(part 1 of 2)
# Autodesk Inventor assembly: Remote_Station
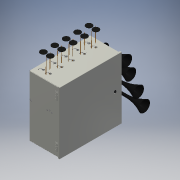
[picture p0: Inventor's stored thumbnail of the model, 180x180]
Saved by Autodesk Inventor 2016 (Build 200138000, 138)
## iProperties
Created: 2016-05-06
Part Number: Remote_Station
Document SubType Name: Assembly
Designer: agmle
Mass: 29128.1 g
Surface Area: 35809.2 cm^2
Volume: 7544.68 cm^3
Density: 3.86075 g/cm^3
Author: agmle
## Documents named in this file (30)
- C:\Users\agmle\BitTorrent Sync\private\projects\Creekfleet_Timer\hardware\CAD\Remote\Remote_Station.iam
- C:\Users\agmle\BitTorrent Sync\private\projects\Creekfleet_Timer\hardware\CAD\Remote\ASM_Winch.iam
- C:\Users\agmle\BitTorrent Sync\private\projects\Creekfleet_Timer\hardware\CAD\Remote\SCESCE-20N2010LP.ipt
- C:\Users\agmle\BitTorrent Sync\private\projects\Creekfleet_Timer\hardware\CAD\Remote\RSF 46-1M_NPT.ipt
- C:\Users\agmle\BitTorrent Sync\private\projects\Creekfleet_Timer\hardware\CAD\Remote\Winch_Plate_Front.ipt
- C:\Users\agmle\Documents\Inventor\Content Center Files\R2016\en-US\ANSI B18.3(05)\ANSI B18.3 - 10-32 UNF - 0.75(31).ipt
- C:\Users\agmle\Documents\Inventor\Content Center Files\R2016\en-US\ANSI B18.22.1\ANSI B18.22.1 - No. 12 - narrow - Type B.ipt
- C:\Users\agmle\Documents\Inventor\Content Center Files\R2016\en-US\ASME B18.21.1(08)\ASME B18.21.1 - No. 12. Carbon Steel(2) A.ipt
- C:\Users\agmle\BitTorrent Sync\private\projects\Creekfleet_Timer\hardware\CAD\Remote\Winch_Plate_Rear.ipt
- C:\Users\agmle\BitTorrent Sync\private\projects\Creekfleet_Timer\hardware\CAD\Remote\Deck_Bushing.iam
- C:\Users\agmle\BitTorrent Sync\private\projects\Creekfleet_Timer\hardware\CAD\Remote\Fender.ipt
- C:\Users\agmle\BitTorrent Sync\private\projects\Creekfleet_Timer\hardware\CAD\Remote\Cherry_KWBH0001\KWBH0001.iam
- C:\Users\agmle\BitTorrent Sync\private\projects\Creekfleet_Timer\hardware\CAD\Remote\Microswitch_Bracket.ipt
- C:\Users\agmle\Documents\Inventor\Content Center Files\R2016\en-US\ASME B18.21.1(08)\ASME B18.21.1 - No. 4. Carbon Steel(2) A.ipt
- C:\Users\agmle\Documents\Inventor\Content Center Files\R2016\en-US\ANSI B18.22.1\ANSI B18.22.1 - No. 4 - narrow - Type B.ipt
- C:\Users\agmle\Documents\Inventor\Content Center Files\R2016\en-US\ANSI B18.3(03)\ANSI B18.3 - 4-40 UNC - UNC - 0.75(1).ipt
- C:\Users\agmle\BitTorrent Sync\private\projects\Creekfleet_Timer\hardware\CAD\Main\9414K360.ipt
- C:\Users\agmle\BitTorrent Sync\private\projects\Creekfleet_Timer\hardware\CAD\Main\9414K930.ipt
- C:\Users\agmle\BitTorrent Sync\private\projects\Creekfleet_Timer\hardware\CAD\Remote\Cap_Mount.ipt
- C:\Users\agmle\BitTorrent Sync\private\projects\Creekfleet_Timer\hardware\CAD\Remote\3.5F_Cap.ipt
- C:\Users\agmle\Documents\Inventor\Content Center Files\R2016\en-US\ANSI B18.3(04)\ANSI B18.3 - 4-40 UNC - 0.25(30).ipt
- C:\Users\agmle\Documents\Inventor\Content Center Files\R2016\en-US\ANSI B18.6.3(36)\ANSI B18.6.3 - 10 - 32(2).ipt
- C:\Users\agmle\BitTorrent Sync\private\projects\Creekfleet_Timer\hardware\CAD\Remote\Horn.iam
- C:\Users\agmle\Documents\Inventor\Content Center Files\R2016\en-US\ANSI B 18.2.4.1 M(1)\ANSI B 18.2.4.1 M - M8 x 1.25Style 1.ipt
- C:\Users\agmle\Documents\Inventor\Content Center Files\R2016\en-US\ANSI B18.22 M\ANSI B18.22M - 8 N.ipt
- C:\Users\agmle\Documents\Inventor\Content Center Files\R2016\en-US\ANSI B18.21.1\ANSI B18.21.1 - 0.375.ipt
- C:\Users\agmle\Documents\Inventor\Content Center Files\R2016\en-US\ANSI B18.2.3.5M\ANSI B18.2.3.5M - M8 x 1.25 x 30.ipt
- C:\Users\agmle\BitTorrent Sync\private\projects\Creekfleet_Timer\hardware\CAD\Remote\Barrel_Jack.ipt
- C:\Users\agmle\BitTorrent Sync\private\projects\Creekfleet_Timer\hardware\CAD\Remote\Norgren-R07-100-RGEA+18-025-003+18-013-212.iam
- C:\Users\agmle\Documents\Inventor\Content Center Files\R2016\en-US\ANSI B18.3(05)\ANSI B18.3 - 10-32 UNF - 0.5(31).ipt
## Components (337 placed, 29 different names)
1. ASM_Winch:1 [sub-assembly] — Insert:6, Insert:7, Insert:93
2. ASM_Winch:2 [sub-assembly] — Insert:5, Insert:8
3. ASM_Winch:3 [sub-assembly] — Insert:4, Insert:9
4. ASM_Winch:4 [sub-assembly] — Insert:3, Insert:10
5. ASM_Winch:5 [sub-assembly] — Insert:2, Insert:11, Insert:92
6. SCESCE-20N2010LP:1 — Insert:1, Insert:12, Insert:13, Insert:26, Insert:27, Insert:28, Insert:29, Insert:30, Insert:31, Insert:98, Insert:99, Insert:104, Insert:105, Insert:106, Insert:107, Insert:108, Insert:109, Insert:110, Insert:111, Insert:112, Insert:113, Insert:114, Insert:115, Mate:1, Mate:2, Mate:3, Mate:4, Mate:5, Mate:6, Mate:7, Mate:8, Mate:9, Mate:10, Mate:11, Mate:12, Flush:1, Mate:14, Angle:1, Mate:16, Mate:17, Insert:147, Insert:148, Mate:18, Mate:19, Mate:20, Mate:21, Mate:22, Mate:23, Mate:24, Mate:25, Mate:26, Mate:27, Mate:28, Mate:29, Mate:30, Mate:31, Mate:32, Mate:33, Mate:34, Mate:35, Insert:248, Insert:249, Insert:250, Insert:251, Insert:252, Insert:253, Insert:254, Insert:255, Insert:256, Insert:257, Insert:258, Insert:259, Insert:260, Insert:261, Insert:262, Insert:263, Insert:264, Insert:265, Insert:267, Insert:268, Insert:269, Insert:286, Insert:287, Insert:288, Insert:289, Insert:294, Mate:47, Insert:304, Insert:305, Insert:306, Insert:307, Mate:48, Insert:308, Tangent:1, Insert:319, Insert:320, Insert:322
7. RSF 46-1M_NPT:1 — Insert:1
8. Winch_Plate_Front:1 — Insert:2, Insert:3, Insert:4, Insert:5, Insert:6, Insert:7, Insert:8, Insert:9, Insert:10, Insert:11, Insert:12, Insert:13, Insert:72, Insert:73, Insert:74, Insert:75, Insert:76, Insert:77, Insert:78, Insert:79, Insert:80, Insert:81, Insert:82, Insert:83, Insert:84, Insert:85, Insert:86, Insert:87, Insert:88, Insert:89, Insert:90, Insert:91
9. Hexagon Socket Head Cap Screw - Inch 10-32 UNF - 0.75:5 — Insert:14
10. Plain Washer (Inch) No. 12 - narrow - Type B:1 — Insert:15, Insert:27
11. Internal Tooth Lock Washer - Type A (Inch) No. 12. Carbon Steel:1 — Insert:14, Insert:15
12. Hexagon Socket Head Cap Screw - Inch 10-32 UNF - 0.75:6
13. Plain Washer (Inch) No. 12 - narrow - Type B:2 — Insert:29
14. Internal Tooth Lock Washer - Type A (Inch) No. 12. Carbon Steel:2
15. Hexagon Socket Head Cap Screw - Inch 10-32 UNF - 0.75:7
16. Plain Washer (Inch) No. 12 - narrow - Type B:3 — Insert:30
17. Internal Tooth Lock Washer - Type A (Inch) No. 12. Carbon Steel:3
18. Hexagon Socket Head Cap Screw - Inch 10-32 UNF - 0.75:8
19. Plain Washer (Inch) No. 12 - narrow - Type B:4 — Insert:26
20. Internal Tooth Lock Washer - Type A (Inch) No. 12. Carbon Steel:4
21. Hexagon Socket Head Cap Screw - Inch 10-32 UNF - 0.75:9
22. Plain Washer (Inch) No. 12 - narrow - Type B:5 — Insert:28
23. Internal Tooth Lock Washer - Type A (Inch) No. 12. Carbon Steel:5
24. Hexagon Socket Head Cap Screw - Inch 10-32 UNF - 0.75:10
25. Plain Washer (Inch) No. 12 - narrow - Type B:6 — Insert:31
26. Internal Tooth Lock Washer - Type A (Inch) No. 12. Carbon Steel:6
27. Hexagon Socket Head Cap Screw - Inch 10-32 UNF - 0.75:11
28. Plain Washer (Inch) No. 12 - narrow - Type B:7 — Insert:72
29. Internal Tooth Lock Washer - Type A (Inch) No. 12. Carbon Steel:7
30. Hexagon Socket Head Cap Screw - Inch 10-32 UNF - 0.75:12
31. Plain Washer (Inch) No. 12 - narrow - Type B:8 — Insert:73
32. Internal Tooth Lock Washer - Type A (Inch) No. 12. Carbon Steel:8
33. Hexagon Socket Head Cap Screw - Inch 10-32 UNF - 0.75:13
34. Plain Washer (Inch) No. 12 - narrow - Type B:9 — Insert:75
35. Internal Tooth Lock Washer - Type A (Inch) No. 12. Carbon Steel:9
36. Hexagon Socket Head Cap Screw - Inch 10-32 UNF - 0.75:14
37. Plain Washer (Inch) No. 12 - narrow - Type B:10 — Insert:74
38. Internal Tooth Lock Washer - Type A (Inch) No. 12. Carbon Steel:10
39. Hexagon Socket Head Cap Screw - Inch 10-32 UNF - 0.75:15
40. Plain Washer (Inch) No. 12 - narrow - Type B:11 — Insert:76
41. Internal Tooth Lock Washer - Type A (Inch) No. 12. Carbon Steel:11
42. Hexagon Socket Head Cap Screw - Inch 10-32 UNF - 0.75:16
43. Plain Washer (Inch) No. 12 - narrow - Type B:12 — Insert:78
44. Internal Tooth Lock Washer - Type A (Inch) No. 12. Carbon Steel:12
45. Hexagon Socket Head Cap Screw - Inch 10-32 UNF - 0.75:17
46. Plain Washer (Inch) No. 12 - narrow - Type B:13 — Insert:79
47. Internal Tooth Lock Washer - Type A (Inch) No. 12. Carbon Steel:13
48. Hexagon Socket Head Cap Screw - Inch 10-32 UNF - 0.75:18
49. Plain Washer (Inch) No. 12 - narrow - Type B:14 — Insert:77
50. Internal Tooth Lock Washer - Type A (Inch) No. 12. Carbon Steel:14
51. Hexagon Socket Head Cap Screw - Inch 10-32 UNF - 0.75:19
52. Plain Washer (Inch) No. 12 - narrow - Type B:15 — Insert:80
53. Internal Tooth Lock Washer - Type A (Inch) No. 12. Carbon Steel:15
54. Hexagon Socket Head Cap Screw - Inch 10-32 UNF - 0.75:20
55. Plain Washer (Inch) No. 12 - narrow - Type B:16 — Insert:81
56. Internal Tooth Lock Washer - Type A (Inch) No. 12. Carbon Steel:16
57. Hexagon Socket Head Cap Screw - Inch 10-32 UNF - 0.75:21
58. Plain Washer (Inch) No. 12 - narrow - Type B:17 — Insert:82
59. Internal Tooth Lock Washer - Type A (Inch) No. 12. Carbon Steel:17
60. Hexagon Socket Head Cap Screw - Inch 10-32 UNF - 0.75:22
61. Plain Washer (Inch) No. 12 - narrow - Type B:18 — Insert:83
62. Internal Tooth Lock Washer - Type A (Inch) No. 12. Carbon Steel:18
63. Hexagon Socket Head Cap Screw - Inch 10-32 UNF - 0.75:23
64. Plain Washer (Inch) No. 12 - narrow - Type B:19 — Insert:84
65. Internal Tooth Lock Washer - Type A (Inch) No. 12. Carbon Steel:19
66. Hexagon Socket Head Cap Screw - Inch 10-32 UNF - 0.75:24
67. Plain Washer (Inch) No. 12 - narrow - Type B:20 — Insert:85
68. Internal Tooth Lock Washer - Type A (Inch) No. 12. Carbon Steel:20
69. Hexagon Socket Head Cap Screw - Inch 10-32 UNF - 0.75:25
70. Plain Washer (Inch) No. 12 - narrow - Type B:21 — Insert:86
71. Internal Tooth Lock Washer - Type A (Inch) No. 12. Carbon Steel:21
72. Hexagon Socket Head Cap Screw - Inch 10-32 UNF - 0.75:26
73. Plain Washer (Inch) No. 12 - narrow - Type B:22 — Insert:87
74. Internal Tooth Lock Washer - Type A (Inch) No. 12. Carbon Steel:22
75. Hexagon Socket Head Cap Screw - Inch 10-32 UNF - 0.75:27
76. Plain Washer (Inch) No. 12 - narrow - Type B:23 — Insert:88
77. Internal Tooth Lock Washer - Type A (Inch) No. 12. Carbon Steel:23
78. Hexagon Socket Head Cap Screw - Inch 10-32 UNF - 0.75:28
79. Plain Washer (Inch) No. 12 - narrow - Type B:24 — Insert:89
80. Internal Tooth Lock Washer - Type A (Inch) No. 12. Carbon Steel:24
81. Hexagon Socket Head Cap Screw - Inch 10-32 UNF - 0.75:29
82. Plain Washer (Inch) No. 12 - narrow - Type B:25 — Insert:90
83. Internal Tooth Lock Washer - Type A (Inch) No. 12. Carbon Steel:25
84. Hexagon Socket Head Cap Screw - Inch 10-32 UNF - 0.75:30
85. Plain Washer (Inch) No. 12 - narrow - Type B:26 — Insert:91
86. Internal Tooth Lock Washer - Type A (Inch) No. 12. Carbon Steel:26
87. Winch_Plate_Rear:1 — Insert:92, Insert:93
88. Hexagon Socket Head Cap Screw - Inch 10-32 UNF - 0.75:31
89. Plain Washer (Inch) No. 12 - narrow - Type B:27 — Insert:98
90. Internal Tooth Lock Washer - Type A (Inch) No. 12. Carbon Steel:27
91. Hexagon Socket Head Cap Screw - Inch 10-32 UNF - 0.75:32
92. Plain Washer (Inch) No. 12 - narrow - Type B:28 — Insert:99
93. Internal Tooth Lock Washer - Type A (Inch) No. 12. Carbon Steel:28
94. Hexagon Socket Head Cap Screw - Inch 10-32 UNF - 0.75:33
95. Plain Washer (Inch) No. 12 - narrow - Type B:29 — Insert:104
96. Internal Tooth Lock Washer - Type A (Inch) No. 12. Carbon Steel:29
97. Hexagon Socket Head Cap Screw - Inch 10-32 UNF - 0.75:34
98. Plain Washer (Inch) No. 12 - narrow - Type B:30 — Insert:105
99. Internal Tooth Lock Washer - Type A (Inch) No. 12. Carbon Steel:30
100. Deck_Bushing:1 [sub-assembly] — Insert:109, Mate:4, Insert:128, Insert:130, Mate:38
101. Deck_Bushing:2 [sub-assembly] — Insert:110, Mate:6, Insert:125, Insert:126, Mate:40
102. Deck_Bushing:3 [sub-assembly] — Insert:107, Mate:2, Insert:132, Insert:134, Mate:36
103. Deck_Bushing:4 [sub-assembly] — Insert:114, Mate:9, Insert:116, Insert:119, Mate:43
104. Deck_Bushing:5 [sub-assembly] — Insert:115, Mate:10, Insert:117, Insert:118, Mate:44
105. Deck_Bushing:6 [sub-assembly] — Insert:111, Mate:5, Insert:124, Insert:127, Mate:39
106. Deck_Bushing:7 [sub-assembly] — Insert:113, Mate:7, Insert:121, Insert:123, Mate:41
107. Deck_Bushing:8 [sub-assembly] — Insert:112, Mate:8, Insert:120, Insert:122, Mate:42
108. Deck_Bushing:9 [sub-assembly] — Insert:106, Mate:1, Insert:133, Insert:135, Mate:13
109. Deck_Bushing:10 [sub-assembly] — Insert:108, Mate:3, Insert:129, Insert:131, Mate:37
110. Hexagon Socket Flat Countersunk Head Cap Screw - Inch 4-40 UNC x 0.25:1 — Insert:116
111. Hexagon Socket Flat Countersunk Head Cap Screw - Inch 4-40 UNC x 0.25:2 — Insert:117
112. Hexagon Socket Flat Countersunk Head Cap Screw - Inch 4-40 UNC x 0.25:3 — Insert:118
113. Hexagon Socket Flat Countersunk Head Cap Screw - Inch 4-40 UNC x 0.25:4 — Insert:120
114. Hexagon Socket Flat Countersunk Head Cap Screw - Inch 4-40 UNC x 0.25:5 — Insert:119
115. Hexagon Socket Flat Countersunk Head Cap Screw - Inch 4-40 UNC x 0.25:6 — Insert:121
116. Hexagon Socket Flat Countersunk Head Cap Screw - Inch 4-40 UNC x 0.25:7 — Insert:123
117. Hexagon Socket Flat Countersunk Head Cap Screw - Inch 4-40 UNC x 0.25:8 — Insert:122
118. Hexagon Socket Flat Countersunk Head Cap Screw - Inch 4-40 UNC x 0.25:9 — Insert:125
119. Hexagon Socket Flat Countersunk Head Cap Screw - Inch 4-40 UNC x 0.25:10 — Insert:124
120. Hexagon Socket Flat Countersunk Head Cap Screw - Inch 4-40 UNC x 0.25:11 — Insert:127
121. Hexagon Socket Flat Countersunk Head Cap Screw - Inch 4-40 UNC x 0.25:12 — Insert:126
122. Hexagon Socket Flat Countersunk Head Cap Screw - Inch 4-40 UNC x 0.25:13 — Insert:129
123. Hexagon Socket Flat Countersunk Head Cap Screw - Inch 4-40 UNC x 0.25:14 — Insert:128
124. Hexagon Socket Flat Countersunk Head Cap Screw - Inch 4-40 UNC x 0.25:15 — Insert:131
125. Hexagon Socket Flat Countersunk Head Cap Screw - Inch 4-40 UNC x 0.25:16 — Insert:130
126. Hexagon Socket Flat Countersunk Head Cap Screw - Inch 4-40 UNC x 0.25:17 — Insert:133
127. Hexagon Socket Flat Countersunk Head Cap Screw - Inch 4-40 UNC x 0.25:18 — Insert:132
128. Hexagon Socket Flat Countersunk Head Cap Screw - Inch 4-40 UNC x 0.25:19 — Insert:135
129. Hexagon Socket Flat Countersunk Head Cap Screw - Inch 4-40 UNC x 0.25:20 — Insert:134
130. Fender:1 — Mate:13, Mate:16, Flush:16
131. KWBH0001:1 [sub-assembly] — Insert:136, Flush:2, Insert:141, Insert:142
132. Microswitch_Bracket:1 — Insert:136, Flush:2, Mate:14, Angle:1, Mate:17, Flush:12
133. Plain Washer (Inch) No. 4 - narrow - Type B:1 — Insert:138, Insert:141
134. Internal Tooth Lock Washer - Type A (Inch) No. 4. Carbon Steel:1 — Insert:138
135. Hexagon Socket Button Head Cap Screw - Inch 4 - 40 - 3/4:1
136. Plain Washer (Inch) No. 4 - narrow - Type B:2 — Insert:142
137. Internal Tooth Lock Washer - Type A (Inch) No. 4. Carbon Steel:2
138. Hexagon Socket Button Head Cap Screw - Inch 4 - 40 - 3/4:2
139. Plain Washer (Inch) No. 4 - narrow - Type B:3 — Insert:147
140. Internal Tooth Lock Washer - Type A (Inch) No. 4. Carbon Steel:3
141. Hexagon Socket Button Head Cap Screw - Inch 4 - 40 - 3/4:3
142. Plain Washer (Inch) No. 4 - narrow - Type B:4 — Insert:148
143. Internal Tooth Lock Washer - Type A (Inch) No. 4. Carbon Steel:4
144. Hexagon Socket Button Head Cap Screw - Inch 4 - 40 - 3/4:4
145. KWBH0001:2 [sub-assembly]
146. Microswitch_Bracket:2 — Mate:18, Mate:29, Flush:13
147. Plain Washer (Inch) No. 4 - narrow - Type B:5
148. Internal Tooth Lock Washer - Type A (Inch) No. 4. Carbon Steel:5
149. Plain Washer (Inch) No. 4 - narrow - Type B:6
150. Internal Tooth Lock Washer - Type A (Inch) No. 4. Carbon Steel:6
151. Hexagon Socket Button Head Cap Screw - Inch 4 - 40 - 3/4:5
152. Hexagon Socket Button Head Cap Screw - Inch 4 - 40 - 3/4:6
153. Plain Washer (Inch) No. 4 - narrow - Type B:7 — Insert:257
154. Internal Tooth Lock Washer - Type A (Inch) No. 4. Carbon Steel:7
155. Hexagon Socket Button Head Cap Screw - Inch 4 - 40 - 3/4:7
156. Plain Washer (Inch) No. 4 - narrow - Type B:8 — Insert:252
157. Internal Tooth Lock Washer - Type A (Inch) No. 4. Carbon Steel:8
158. Hexagon Socket Button Head Cap Screw - Inch 4 - 40 - 3/4:8
159. KWBH0001:3 [sub-assembly]
160. Microswitch_Bracket:3 — Mate:22, Mate:30, Flush:14
161. Plain Washer (Inch) No. 4 - narrow - Type B:9
162. Internal Tooth Lock Washer - Type A (Inch) No. 4. Carbon Steel:9
163. Plain Washer (Inch) No. 4 - narrow - Type B:10
164. Internal Tooth Lock Washer - Type A (Inch) No. 4. Carbon Steel:10
165. Hexagon Socket Button Head Cap Screw - Inch 4 - 40 - 3/4:9
166. Hexagon Socket Button Head Cap Screw - Inch 4 - 40 - 3/4:10
167. Plain Washer (Inch) No. 4 - narrow - Type B:11 — Insert:258
168. Internal Tooth Lock Washer - Type A (Inch) No. 4. Carbon Steel:11
169. Hexagon Socket Button Head Cap Screw - Inch 4 - 40 - 3/4:11
170. Plain Washer (Inch) No. 4 - narrow - Type B:12 — Insert:256
171. Internal Tooth Lock Washer - Type A (Inch) No. 4. Carbon Steel:12
172. Hexagon Socket Button Head Cap Screw - Inch 4 - 40 - 3/4:12
173. KWBH0001:4 [sub-assembly]
174. Microswitch_Bracket:4 — Mate:24, Mate:33, Flush:15
175. Plain Washer (Inch) No. 4 - narrow - Type B:13
176. Internal Tooth Lock Washer - Type A (Inch) No. 4. Carbon Steel:13
177. Plain Washer (Inch) No. 4 - narrow - Type B:14
178. Internal Tooth Lock Washer - Type A (Inch) No. 4. Carbon Steel:14
179. Hexagon Socket Button Head Cap Screw - Inch 4 - 40 - 3/4:13
180. Hexagon Socket Button Head Cap Screw - Inch 4 - 40 - 3/4:14
181. Plain Washer (Inch) No. 4 - narrow - Type B:15 — Insert:261
182. Internal Tooth Lock Washer - Type A (Inch) No. 4. Carbon Steel:15
183. Hexagon Socket Button Head Cap Screw - Inch 4 - 40 - 3/4:15
184. Plain Washer (Inch) No. 4 - narrow - Type B:16 — Insert:260
185. Internal Tooth Lock Washer - Type A (Inch) No. 4. Carbon Steel:16
186. Hexagon Socket Button Head Cap Screw - Inch 4 - 40 - 3/4:16
187. KWBH0001:5 [sub-assembly]
188. Microswitch_Bracket:5 — Mate:26, Mate:34
189. Plain Washer (Inch) No. 4 - narrow - Type B:17
190. Internal Tooth Lock Washer - Type A (Inch) No. 4. Carbon Steel:17
191. Plain Washer (Inch) No. 4 - narrow - Type B:18
192. Internal Tooth Lock Washer - Type A (Inch) No. 4. Carbon Steel:18
193. Hexagon Socket Button Head Cap Screw - Inch 4 - 40 - 3/4:17
194. Hexagon Socket Button Head Cap Screw - Inch 4 - 40 - 3/4:18
195. Plain Washer (Inch) No. 4 - narrow - Type B:19 — Insert:264
196. Internal Tooth Lock Washer - Type A (Inch) No. 4. Carbon Steel:19
197. Hexagon Socket Button Head Cap Screw - Inch 4 - 40 - 3/4:19
198. Plain Washer (Inch) No. 4 - narrow - Type B:20 — Insert:265
199. Internal Tooth Lock Washer - Type A (Inch) No. 4. Carbon Steel:20
200. Hexagon Socket Button Head Cap Screw - Inch 4 - 40 - 3/4:20
201. KWBH0001:6 [sub-assembly]
202. Microswitch_Bracket:6 — Mate:19, Mate:27, Flush:12
203. Plain Washer (Inch) No. 4 - narrow - Type B:21
204. Internal Tooth Lock Washer - Type A (Inch) No. 4. Carbon Steel:21
205. Plain Washer (Inch) No. 4 - narrow - Type B:22
206. Internal Tooth Lock Washer - Type A (Inch) No. 4. Carbon Steel:22
207. Hexagon Socket Button Head Cap Screw - Inch 4 - 40 - 3/4:21
208. Hexagon Socket Button Head Cap Screw - Inch 4 - 40 - 3/4:22
209. Plain Washer (Inch) No. 4 - narrow - Type B:23 — Insert:249
210. Internal Tooth Lock Washer - Type A (Inch) No. 4. Carbon Steel:23
211. Hexagon Socket Button Head Cap Screw - Inch 4 - 40 - 3/4:23
212. Plain Washer (Inch) No. 4 - narrow - Type B:24 — Insert:248
213. Internal Tooth Lock Washer - Type A (Inch) No. 4. Carbon Steel:24
214. Hexagon Socket Button Head Cap Screw - Inch 4 - 40 - 3/4:24
215. KWBH0001:7 [sub-assembly]
216. Microswitch_Bracket:7 — Mate:20, Mate:28, Flush:13
217. Plain Washer (Inch) No. 4 - narrow - Type B:25
218. Internal Tooth Lock Washer - Type A (Inch) No. 4. Carbon Steel:25
219. Plain Washer (Inch) No. 4 - narrow - Type B:26
220. Internal Tooth Lock Washer - Type A (Inch) No. 4. Carbon Steel:26
221. Hexagon Socket Button Head Cap Screw - Inch 4 - 40 - 3/4:25
222. Hexagon Socket Button Head Cap Screw - Inch 4 - 40 - 3/4:26
223. Plain Washer (Inch) No. 4 - narrow - Type B:27 — Insert:251
224. Internal Tooth Lock Washer - Type A (Inch) No. 4. Carbon Steel:27
225. Hexagon Socket Button Head Cap Screw - Inch 4 - 40 - 3/4:27
226. Plain Washer (Inch) No. 4 - narrow - Type B:28 — Insert:250
227. Internal Tooth Lock Washer - Type A (Inch) No. 4. Carbon Steel:28
228. Hexagon Socket Button Head Cap Screw - Inch 4 - 40 - 3/4:28
229. KWBH0001:8 [sub-assembly]
230. Microswitch_Bracket:8 — Mate:21, Mate:31, Flush:14
231. Plain Washer (Inch) No. 4 - narrow - Type B:29
232. Internal Tooth Lock Washer - Type A (Inch) No. 4. Carbon Steel:29
233. Plain Washer (Inch) No. 4 - narrow - Type B:30
234. Internal Tooth Lock Washer - Type A (Inch) No. 4. Carbon Steel:30
235. Hexagon Socket Button Head Cap Screw - Inch 4 - 40 - 3/4:29
236. Hexagon Socket Button Head Cap Screw - Inch 4 - 40 - 3/4:30
237. Plain Washer (Inch) No. 4 - narrow - Type B:31 — Insert:254
238. Internal Tooth Lock Washer - Type A (Inch) No. 4. Carbon Steel:31
239. Hexagon Socket Button Head Cap Screw - Inch 4 - 40 - 3/4:31
240. Plain Washer (Inch) No. 4 - narrow - Type B:32 — Insert:253
241. Internal Tooth Lock Washer - Type A (Inch) No. 4. Carbon Steel:32
242. Hexagon Socket Button Head Cap Screw - Inch 4 - 40 - 3/4:32
243. KWBH0001:9 [sub-assembly]
244. Microswitch_Bracket:9 — Mate:23, Mate:32, Flush:15
245. Plain Washer (Inch) No. 4 - narrow - Type B:33
246. Internal Tooth Lock Washer - Type A (Inch) No. 4. Carbon Steel:33
247. Plain Washer (Inch) No. 4 - narrow - Type B:34
248. Internal Tooth Lock Washer - Type A (Inch) No. 4. Carbon Steel:34
249. Hexagon Socket Button Head Cap Screw - Inch 4 - 40 - 3/4:33
250. Hexagon Socket Button Head Cap Screw - Inch 4 - 40 - 3/4:34
251. Plain Washer (Inch) No. 4 - narrow - Type B:35 — Insert:259
252. Internal Tooth Lock Washer - Type A (Inch) No. 4. Carbon Steel:35
253. Hexagon Socket Button Head Cap Screw - Inch 4 - 40 - 3/4:35
254. Plain Washer (Inch) No. 4 - narrow - Type B:36 — Insert:255
255. Internal Tooth Lock Washer - Type A (Inch) No. 4. Carbon Steel:36
256. Hexagon Socket Button Head Cap Screw - Inch 4 - 40 - 3/4:36
257. KWBH0001:10 [sub-assembly]
258. Microswitch_Bracket:10 — Mate:25, Mate:35
259. Plain Washer (Inch) No. 4 - narrow - Type B:37
260. Internal Tooth Lock Washer - Type A (Inch) No. 4. Carbon Steel:37
261. Plain Washer (Inch) No. 4 - narrow - Type B:38
262. Internal Tooth Lock Washer - Type A (Inch) No. 4. Carbon Steel:38
263. Hexagon Socket Button Head Cap Screw - Inch 4 - 40 - 3/4:37
264. Hexagon Socket Button Head Cap Screw - Inch 4 - 40 - 3/4:38
265. Plain Washer (Inch) No. 4 - narrow - Type B:39 — Insert:263
266. Internal Tooth Lock Washer - Type A (Inch) No. 4. Carbon Steel:39
267. Hexagon Socket Button Head Cap Screw - Inch 4 - 40 - 3/4:39
268. Plain Washer (Inch) No. 4 - narrow - Type B:40 — Insert:262
269. Internal Tooth Lock Washer - Type A (Inch) No. 4. Carbon Steel:40
270. Hexagon Socket Button Head Cap Screw - Inch 4 - 40 - 3/4:40
271. Fender:2 — Mate:39, Flush:17, Flush:18
272. Fender:3 — Mate:40, Flush:22, Flush:23
273. Fender:4 — Mate:41, Flush:18, Flush:19
274. Fender:5 — Mate:43, Flush:19, Flush:20
275. Fender:6 — Mate:36, Flush:24
276. Fender:7 — Mate:37, Flush:16, Flush:17
277. Fender:8 — Mate:38, Flush:23, Flush:24
278. Fender:9 — Mate:42, Flush:21, Flush:22
279. Fender:10 — Mate:44, Flush:20, Flush:21
280. 9414K360:1 — Insert:266
281. 9414K930:1 — Insert:266, Insert:267
282. Cap_Mount:1 — Mate:46, Insert:268, Insert:280, Insert:281
283. Cap_Mount:2 — Mate:45, Insert:269, Insert:278, Insert:279, Flush:25
284. 3.5F_Cap:1 — Mate:45, Mate:46, Flush:25
285. Hexagon Socket Head Cap Screw - Inch 10-32 UNF - 0.5:6
286. Plain Washer (Inch) No. 12 - narrow - Type B:31 — Insert:278
287. Internal Tooth Lock Washer - Type A (Inch) No. 12. Carbon Steel:31
288. Hexagon Socket Head Cap Screw - Inch 10-32 UNF - 0.5:4
289. Plain Washer (Inch) No. 12 - narrow - Type B:32 — Insert:281
290. Internal Tooth Lock Washer - Type A (Inch) No. 12. Carbon Steel:32
291. Hexagon Socket Head Cap Screw - Inch 10-32 UNF - 0.5:3
292. Plain Washer (Inch) No. 12 - narrow - Type B:33 — Insert:280
293. Internal Tooth Lock Washer - Type A (Inch) No. 12. Carbon Steel:33
294. Hexagon Socket Head Cap Screw - Inch 10-32 UNF - 0.5:5
295. Plain Washer (Inch) No. 12 - narrow - Type B:34 — Insert:279
296. Internal Tooth Lock Washer - Type A (Inch) No. 12. Carbon Steel:34
297. Plain Washer (Inch) No. 12 - narrow - Type B:35 — Insert:286
298. Internal Tooth Lock Washer - Type A (Inch) No. 12. Carbon Steel:35 — Insert:292
299. Plain Washer (Inch) No. 12 - narrow - Type B:36 — Insert:289
300. Internal Tooth Lock Washer - Type A (Inch) No. 12. Carbon Steel:36 — Insert:290
301. Plain Washer (Inch) No. 12 - narrow - Type B:37 — Insert:287
302. Internal Tooth Lock Washer - Type A (Inch) No. 12. Carbon Steel:37 — Insert:293
303. Plain Washer (Inch) No. 12 - narrow - Type B:38 — Insert:288
304. Internal Tooth Lock Washer - Type A (Inch) No. 12. Carbon Steel:38 — Insert:291
305. Hex Machine Screw Nut - Inch 10 - 32:1 — Insert:290
306. Hex Machine Screw Nut - Inch 10 - 32:2 — Insert:291
307. Hex Machine Screw Nut - Inch 10 - 32:3 — Insert:292
308. Hex Machine Screw Nut - Inch 10 - 32:4 — Insert:293
309. Horn:1 [sub-assembly] — Insert:294, Mate:47, Insert:301, Insert:302, Insert:303
310. Hex Nut Metric M8 x 1.25:1 — Insert:299
311. Hex Nut Metric M8 x 1.25:2 — Insert:298
312. Hex Nut Metric M8 x 1.25:3 — Insert:300
313. Plain Washer (Metric) 8 N:1 — Insert:295, Insert:302
314. Plain Washer (Metric) 8 N:2 — Insert:296, Insert:301
315. Plain Washer (Metric) 8 N:3 — Insert:297, Insert:303
316. Helical Spring Lock Washers 0.375:1 — Insert:298, Insert:304
317. Helical Spring Lock Washers 0.375:2 — Insert:299, Insert:305
318. Helical Spring Lock Washers 0.375:3 — Insert:300, Insert:306
319. Hex Bolt - Metric M8 x 1.25 x 30:1 — Insert:295
320. Hex Bolt - Metric M8 x 1.25 x 30:2 — Insert:296
321. Hex Bolt - Metric M8 x 1.25 x 30:3 — Insert:297
322. Barrel_Jack:1 — Insert:307, Mate:48
323. Norgren-R07-100-RGEA+18-025-003+18-013-212:1 [sub-assembly] — Insert:308, Tangent:1, Insert:317, Insert:318
324. Hexagon Socket Head Cap Screw - Inch 10-32 UNF - 0.5:2
325. Plain Washer (Inch) No. 12 - narrow - Type B:39 — Insert:318
326. Internal Tooth Lock Washer - Type A (Inch) No. 12. Carbon Steel:39
327. Plain Washer (Inch) No. 12 - narrow - Type B:40 — Insert:320
328. Internal Tooth Lock Washer - Type A (Inch) No. 12. Carbon Steel:40
329. Hex Machine Screw Nut - Inch 10 - 32:5
330. Hexagon Socket Head Cap Screw - Inch 10-32 UNF - 0.5:1
331. Plain Washer (Inch) No. 12 - narrow - Type B:41 — Insert:317
332. Internal Tooth Lock Washer - Type A (Inch) No. 12. Carbon Steel:41
333. Plain Washer (Inch) No. 12 - narrow - Type B:42 — Insert:319
334. Internal Tooth Lock Washer - Type A (Inch) No. 12. Carbon Steel:42
335. Hex Machine Screw Nut - Inch 10 - 32:6
336. 9414K360:2
337. 9414K930:2 — Insert:322
## Relationships (396: Insert 322, Mate 47, Flush 25, Angle 1, Tangent 1)
- Insert:1: SCESCE-20N2010LP:1 ↔ RSF 46-1M_NPT:1
- Insert:2: ASM_Winch:5 ↔ Winch_Plate_Front:1
- Insert:3: ASM_Winch:4 ↔ Winch_Plate_Front:1
- Insert:4: ASM_Winch:3 ↔ Winch_Plate_Front:1
- Insert:5: ASM_Winch:2 ↔ Winch_Plate_Front:1
- Insert:6: ASM_Winch:1 ↔ Winch_Plate_Front:1
- Insert:7: ASM_Winch:1 ↔ Winch_Plate_Front:1
- Insert:8: ASM_Winch:2 ↔ Winch_Plate_Front:1
- Insert:9: ASM_Winch:3 ↔ Winch_Plate_Front:1
- Insert:10: ASM_Winch:4 ↔ Winch_Plate_Front:1
- Insert:11: ASM_Winch:5 ↔ Winch_Plate_Front:1
- Insert:12: SCESCE-20N2010LP:1 ↔ Winch_Plate_Front:1
- Insert:13: SCESCE-20N2010LP:1 ↔ Winch_Plate_Front:1
- Insert:14: Hexagon Socket Head Cap Screw - Inch 10-32 UNF - 0.75:5 ↔ Internal Tooth Lock Washer - Type A (Inch) No. 12. Carbon Steel:1
- Insert:15: Plain Washer (Inch) No. 12 - narrow - Type B:1 ↔ Internal Tooth Lock Washer - Type A (Inch) No. 12. Carbon Steel:1
- [Insert]: Hexagon Socket Head Cap Screw - Inch 10-32 UNF - 0.75:6 ↔ Internal Tooth Lock Washer - Type A (Inch) No. 12. Carbon Steel:2
- [Insert]: Plain Washer (Inch) No. 12 - narrow - Type B:2 ↔ Internal Tooth Lock Washer - Type A (Inch) No. 12. Carbon Steel:2
- [Insert]: Hexagon Socket Head Cap Screw - Inch 10-32 UNF - 0.75:7 ↔ Internal Tooth Lock Washer - Type A (Inch) No. 12. Carbon Steel:3
- [Insert]: Plain Washer (Inch) No. 12 - narrow - Type B:3 ↔ Internal Tooth Lock Washer - Type A (Inch) No. 12. Carbon Steel:3
- [Insert]: Hexagon Socket Head Cap Screw - Inch 10-32 UNF - 0.75:8 ↔ Internal Tooth Lock Washer - Type A (Inch) No. 12. Carbon Steel:4
- [Insert]: Plain Washer (Inch) No. 12 - narrow - Type B:4 ↔ Internal Tooth Lock Washer - Type A (Inch) No. 12. Carbon Steel:4
- [Insert]: Hexagon Socket Head Cap Screw - Inch 10-32 UNF - 0.75:9 ↔ Internal Tooth Lock Washer - Type A (Inch) No. 12. Carbon Steel:5
- [Insert]: Plain Washer (Inch) No. 12 - narrow - Type B:5 ↔ Internal Tooth Lock Washer - Type A (Inch) No. 12. Carbon Steel:5
- [Insert]: Hexagon Socket Head Cap Screw - Inch 10-32 UNF - 0.75:10 ↔ Internal Tooth Lock Washer - Type A (Inch) No. 12. Carbon Steel:6
- [Insert]: Plain Washer (Inch) No. 12 - narrow - Type B:6 ↔ Internal Tooth Lock Washer - Type A (Inch) No. 12. Carbon Steel:6
- Insert:26: SCESCE-20N2010LP:1 ↔ Plain Washer (Inch) No. 12 - narrow - Type B:4
- Insert:27: SCESCE-20N2010LP:1 ↔ Plain Washer (Inch) No. 12 - narrow - Type B:1
- Insert:28: SCESCE-20N2010LP:1 ↔ Plain Washer (Inch) No. 12 - narrow - Type B:5
- Insert:29: SCESCE-20N2010LP:1 ↔ Plain Washer (Inch) No. 12 - narrow - Type B:2
- Insert:30: SCESCE-20N2010LP:1 ↔ Plain Washer (Inch) No. 12 - narrow - Type B:3
- Insert:31: SCESCE-20N2010LP:1 ↔ Plain Washer (Inch) No. 12 - narrow - Type B:6
- [Insert]: Hexagon Socket Head Cap Screw - Inch 10-32 UNF - 0.75:11 ↔ Internal Tooth Lock Washer - Type A (Inch) No. 12. Carbon Steel:7
- [Insert]: Plain Washer (Inch) No. 12 - narrow - Type B:7 ↔ Internal Tooth Lock Washer - Type A (Inch) No. 12. Carbon Steel:7
- [Insert]: Hexagon Socket Head Cap Screw - Inch 10-32 UNF - 0.75:12 ↔ Internal Tooth Lock Washer - Type A (Inch) No. 12. Carbon Steel:8
- [Insert]: Plain Washer (Inch) No. 12 - narrow - Type B:8 ↔ Internal Tooth Lock Washer - Type A (Inch) No. 12. Carbon Steel:8
- [Insert]: Hexagon Socket Head Cap Screw - Inch 10-32 UNF - 0.75:13 ↔ Internal Tooth Lock Washer - Type A (Inch) No. 12. Carbon Steel:9
- [Insert]: Plain Washer (Inch) No. 12 - narrow - Type B:9 ↔ Internal Tooth Lock Washer - Type A (Inch) No. 12. Carbon Steel:9
- [Insert]: Hexagon Socket Head Cap Screw - Inch 10-32 UNF - 0.75:14 ↔ Internal Tooth Lock Washer - Type A (Inch) No. 12. Carbon Steel:10
- [Insert]: Plain Washer (Inch) No. 12 - narrow - Type B:10 ↔ Internal Tooth Lock Washer - Type A (Inch) No. 12. Carbon Steel:10
- [Insert]: Hexagon Socket Head Cap Screw - Inch 10-32 UNF - 0.75:15 ↔ Internal Tooth Lock Washer - Type A (Inch) No. 12. Carbon Steel:11
- [Insert]: Plain Washer (Inch) No. 12 - narrow - Type B:11 ↔ Internal Tooth Lock Washer - Type A (Inch) No. 12. Carbon Steel:11
- [Insert]: Hexagon Socket Head Cap Screw - Inch 10-32 UNF - 0.75:16 ↔ Internal Tooth Lock Washer - Type A (Inch) No. 12. Carbon Steel:12
- [Insert]: Plain Washer (Inch) No. 12 - narrow - Type B:12 ↔ Internal Tooth Lock Washer - Type A (Inch) No. 12. Carbon Steel:12
- [Insert]: Hexagon Socket Head Cap Screw - Inch 10-32 UNF - 0.75:17 ↔ Internal Tooth Lock Washer - Type A (Inch) No. 12. Carbon Steel:13
- [Insert]: Plain Washer (Inch) No. 12 - narrow - Type B:13 ↔ Internal Tooth Lock Washer - Type A (Inch) No. 12. Carbon Steel:13
- [Insert]: Hexagon Socket Head Cap Screw - Inch 10-32 UNF - 0.75:18 ↔ Internal Tooth Lock Washer - Type A (Inch) No. 12. Carbon Steel:14
- [Insert]: Plain Washer (Inch) No. 12 - narrow - Type B:14 ↔ Internal Tooth Lock Washer - Type A (Inch) No. 12. Carbon Steel:14
- [Insert]: Hexagon Socket Head Cap Screw - Inch 10-32 UNF - 0.75:19 ↔ Internal Tooth Lock Washer - Type A (Inch) No. 12. Carbon Steel:15
- [Insert]: Plain Washer (Inch) No. 12 - narrow - Type B:15 ↔ Internal Tooth Lock Washer - Type A (Inch) No. 12. Carbon Steel:15
- [Insert]: Hexagon Socket Head Cap Screw - Inch 10-32 UNF - 0.75:20 ↔ Internal Tooth Lock Washer - Type A (Inch) No. 12. Carbon Steel:16
- [Insert]: Plain Washer (Inch) No. 12 - narrow - Type B:16 ↔ Internal Tooth Lock Washer - Type A (Inch) No. 12. Carbon Steel:16
- [Insert]: Hexagon Socket Head Cap Screw - Inch 10-32 UNF - 0.75:21 ↔ Internal Tooth Lock Washer - Type A (Inch) No. 12. Carbon Steel:17
- [Insert]: Plain Washer (Inch) No. 12 - narrow - Type B:17 ↔ Internal Tooth Lock Washer - Type A (Inch) No. 12. Carbon Steel:17
- [Insert]: Hexagon Socket Head Cap Screw - Inch 10-32 UNF - 0.75:22 ↔ Internal Tooth Lock Washer - Type A (Inch) No. 12. Carbon Steel:18
- [Insert]: Plain Washer (Inch) No. 12 - narrow - Type B:18 ↔ Internal Tooth Lock Washer - Type A (Inch) No. 12. Carbon Steel:18
- [Insert]: Hexagon Socket Head Cap Screw - Inch 10-32 UNF - 0.75:23 ↔ Internal Tooth Lock Washer - Type A (Inch) No. 12. Carbon Steel:19
- [Insert]: Plain Washer (Inch) No. 12 - narrow - Type B:19 ↔ Internal Tooth Lock Washer - Type A (Inch) No. 12. Carbon Steel:19
- [Insert]: Hexagon Socket Head Cap Screw - Inch 10-32 UNF - 0.75:24 ↔ Internal Tooth Lock Washer - Type A (Inch) No. 12. Carbon Steel:20
- [Insert]: Plain Washer (Inch) No. 12 - narrow - Type B:20 ↔ Internal Tooth Lock Washer - Type A (Inch) No. 12. Carbon Steel:20
- [Insert]: Hexagon Socket Head Cap Screw - Inch 10-32 UNF - 0.75:25 ↔ Internal Tooth Lock Washer - Type A (Inch) No. 12. Carbon Steel:21
- [Insert]: Plain Washer (Inch) No. 12 - narrow - Type B:21 ↔ Internal Tooth Lock Washer - Type A (Inch) No. 12. Carbon Steel:21
- [Insert]: Hexagon Socket Head Cap Screw - Inch 10-32 UNF - 0.75:26 ↔ Internal Tooth Lock Washer - Type A (Inch) No. 12. Carbon Steel:22
- [Insert]: Plain Washer (Inch) No. 12 - narrow - Type B:22 ↔ Internal Tooth Lock Washer - Type A (Inch) No. 12. Carbon Steel:22
- [Insert]: Hexagon Socket Head Cap Screw - Inch 10-32 UNF - 0.75:27 ↔ Internal Tooth Lock Washer - Type A (Inch) No. 12. Carbon Steel:23
- [Insert]: Plain Washer (Inch) No. 12 - narrow - Type B:23 ↔ Internal Tooth Lock Washer - Type A (Inch) No. 12. Carbon Steel:23
- [Insert]: Hexagon Socket Head Cap Screw - Inch 10-32 UNF - 0.75:28 ↔ Internal Tooth Lock Washer - Type A (Inch) No. 12. Carbon Steel:24
- [Insert]: Plain Washer (Inch) No. 12 - narrow - Type B:24 ↔ Internal Tooth Lock Washer - Type A (Inch) No. 12. Carbon Steel:24
- [Insert]: Hexagon Socket Head Cap Screw - Inch 10-32 UNF - 0.75:29 ↔ Internal Tooth Lock Washer - Type A (Inch) No. 12. Carbon Steel:25
- [Insert]: Plain Washer (Inch) No. 12 - narrow - Type B:25 ↔ Internal Tooth Lock Washer - Type A (Inch) No. 12. Carbon Steel:25
- [Insert]: Hexagon Socket Head Cap Screw - Inch 10-32 UNF - 0.75:30 ↔ Internal Tooth Lock Washer - Type A (Inch) No. 12. Carbon Steel:26
- [Insert]: Plain Washer (Inch) No. 12 - narrow - Type B:26 ↔ Internal Tooth Lock Washer - Type A (Inch) No. 12. Carbon Steel:26
- Insert:72: Winch_Plate_Front:1 ↔ Plain Washer (Inch) No. 12 - narrow - Type B:7
- Insert:73: Winch_Plate_Front:1 ↔ Plain Washer (Inch) No. 12 - narrow - Type B:8
- Insert:74: Winch_Plate_Front:1 ↔ Plain Washer (Inch) No. 12 - narrow - Type B:10
- Insert:75: Winch_Plate_Front:1 ↔ Plain Washer (Inch) No. 12 - narrow - Type B:9
- Insert:76: Winch_Plate_Front:1 ↔ Plain Washer (Inch) No. 12 - narrow - Type B:11
- Insert:77: Winch_Plate_Front:1 ↔ Plain Washer (Inch) No. 12 - narrow - Type B:14
- Insert:78: Winch_Plate_Front:1 ↔ Plain Washer (Inch) No. 12 - narrow - Type B:12
- Insert:79: Winch_Plate_Front:1 ↔ Plain Washer (Inch) No. 12 - narrow - Type B:13
- Insert:80: Winch_Plate_Front:1 ↔ Plain Washer (Inch) No. 12 - narrow - Type B:15
- Insert:81: Winch_Plate_Front:1 ↔ Plain Washer (Inch) No. 12 - narrow - Type B:16
- Insert:82: Winch_Plate_Front:1 ↔ Plain Washer (Inch) No. 12 - narrow - Type B:17
- Insert:83: Winch_Plate_Front:1 ↔ Plain Washer (Inch) No. 12 - narrow - Type B:18
- Insert:84: Winch_Plate_Front:1 ↔ Plain Washer (Inch) No. 12 - narrow - Type B:19
- Insert:85: Winch_Plate_Front:1 ↔ Plain Washer (Inch) No. 12 - narrow - Type B:20
- Insert:86: Winch_Plate_Front:1 ↔ Plain Washer (Inch) No. 12 - narrow - Type B:21
- Insert:87: Winch_Plate_Front:1 ↔ Plain Washer (Inch) No. 12 - narrow - Type B:22
- Insert:88: Winch_Plate_Front:1 ↔ Plain Washer (Inch) No. 12 - narrow - Type B:23
- Insert:89: Winch_Plate_Front:1 ↔ Plain Washer (Inch) No. 12 - narrow - Type B:24
- Insert:90: Winch_Plate_Front:1 ↔ Plain Washer (Inch) No. 12 - narrow - Type B:25
- Insert:91: Winch_Plate_Front:1 ↔ Plain Washer (Inch) No. 12 - narrow - Type B:26
- Insert:92: ASM_Winch:5 ↔ Winch_Plate_Rear:1
- Insert:93: ASM_Winch:1 ↔ Winch_Plate_Rear:1
- [Insert]: Hexagon Socket Head Cap Screw - Inch 10-32 UNF - 0.75:31 ↔ Internal Tooth Lock Washer - Type A (Inch) No. 12. Carbon Steel:27
- [Insert]: Plain Washer (Inch) No. 12 - narrow - Type B:27 ↔ Internal Tooth Lock Washer - Type A (Inch) No. 12. Carbon Steel:27
- [Insert]: Hexagon Socket Head Cap Screw - Inch 10-32 UNF - 0.75:32 ↔ Internal Tooth Lock Washer - Type A (Inch) No. 12. Carbon Steel:28
- [Insert]: Plain Washer (Inch) No. 12 - narrow - Type B:28 ↔ Internal Tooth Lock Washer - Type A (Inch) No. 12. Carbon Steel:28
- Insert:98: SCESCE-20N2010LP:1 ↔ Plain Washer (Inch) No. 12 - narrow - Type B:27
- Insert:99: SCESCE-20N2010LP:1 ↔ Plain Washer (Inch) No. 12 - narrow - Type B:28
- [Insert]: Hexagon Socket Head Cap Screw - Inch 10-32 UNF - 0.75:33 ↔ Internal Tooth Lock Washer - Type A (Inch) No. 12. Carbon Steel:29
- [Insert]: Plain Washer (Inch) No. 12 - narrow - Type B:29 ↔ Internal Tooth Lock Washer - Type A (Inch) No. 12. Carbon Steel:29
- [Insert]: Hexagon Socket Head Cap Screw - Inch 10-32 UNF - 0.75:34 ↔ Internal Tooth Lock Washer - Type A (Inch) No. 12. Carbon Steel:30
- [Insert]: Plain Washer (Inch) No. 12 - narrow - Type B:30 ↔ Internal Tooth Lock Washer - Type A (Inch) No. 12. Carbon Steel:30
- Insert:104: SCESCE-20N2010LP:1 ↔ Plain Washer (Inch) No. 12 - narrow - Type B:29
- Insert:105: SCESCE-20N2010LP:1 ↔ Plain Washer (Inch) No. 12 - narrow - Type B:30
- Insert:106: SCESCE-20N2010LP:1 ↔ Deck_Bushing:9
- Insert:107: SCESCE-20N2010LP:1 ↔ Deck_Bushing:3
- Insert:108: SCESCE-20N2010LP:1 ↔ Deck_Bushing:10
- Insert:109: SCESCE-20N2010LP:1 ↔ Deck_Bushing:1
- Insert:110: SCESCE-20N2010LP:1 ↔ Deck_Bushing:2
- Insert:111: SCESCE-20N2010LP:1 ↔ Deck_Bushing:6
- Insert:112: SCESCE-20N2010LP:1 ↔ Deck_Bushing:8
- Insert:113: SCESCE-20N2010LP:1 ↔ Deck_Bushing:7
- Insert:114: SCESCE-20N2010LP:1 ↔ Deck_Bushing:4
- Insert:115: SCESCE-20N2010LP:1 ↔ Deck_Bushing:5
- Mate:1: SCESCE-20N2010LP:1 ↔ Deck_Bushing:9
- Mate:2: SCESCE-20N2010LP:1 ↔ Deck_Bushing:3
- Mate:3: SCESCE-20N2010LP:1 ↔ Deck_Bushing:10
- Mate:4: SCESCE-20N2010LP:1 ↔ Deck_Bushing:1
- Mate:5: SCESCE-20N2010LP:1 ↔ Deck_Bushing:6
- Mate:6: SCESCE-20N2010LP:1 ↔ Deck_Bushing:2
- Mate:7: SCESCE-20N2010LP:1 ↔ Deck_Bushing:7
- Mate:8: SCESCE-20N2010LP:1 ↔ Deck_Bushing:8
- Mate:9: SCESCE-20N2010LP:1 ↔ Deck_Bushing:4
- Mate:10: SCESCE-20N2010LP:1 ↔ Deck_Bushing:5
- Mate:11: SCESCE-20N2010LP:1
- Mate:12: SCESCE-20N2010LP:1
- Flush:1: SCESCE-20N2010LP:1
- Insert:116: Deck_Bushing:4 ↔ Hexagon Socket Flat Countersunk Head Cap Screw - Inch 4-40 UNC x 0.25:1
- Insert:117: Deck_Bushing:5 ↔ Hexagon Socket Flat Countersunk Head Cap Screw - Inch 4-40 UNC x 0.25:2
- Insert:118: Deck_Bushing:5 ↔ Hexagon Socket Flat Countersunk Head Cap Screw - Inch 4-40 UNC x 0.25:3
- Insert:119: Deck_Bushing:4 ↔ Hexagon Socket Flat Countersunk Head Cap Screw - Inch 4-40 UNC x 0.25:5
- Insert:120: Deck_Bushing:8 ↔ Hexagon Socket Flat Countersunk Head Cap Screw - Inch 4-40 UNC x 0.25:4
- Insert:121: Deck_Bushing:7 ↔ Hexagon Socket Flat Countersunk Head Cap Screw - Inch 4-40 UNC x 0.25:6
- Insert:122: Deck_Bushing:8 ↔ Hexagon Socket Flat Countersunk Head Cap Screw - Inch 4-40 UNC x 0.25:8
- Insert:123: Deck_Bushing:7 ↔ Hexagon Socket Flat Countersunk Head Cap Screw - Inch 4-40 UNC x 0.25:7
- Insert:124: Deck_Bushing:6 ↔ Hexagon Socket Flat Countersunk Head Cap Screw - Inch 4-40 UNC x 0.25:10
- Insert:125: Deck_Bushing:2 ↔ Hexagon Socket Flat Countersunk Head Cap Screw - Inch 4-40 UNC x 0.25:9
- Insert:126: Deck_Bushing:2 ↔ Hexagon Socket Flat Countersunk Head Cap Screw - Inch 4-40 UNC x 0.25:12
- Insert:127: Deck_Bushing:6 ↔ Hexagon Socket Flat Countersunk Head Cap Screw - Inch 4-40 UNC x 0.25:11
- Insert:128: Deck_Bushing:1 ↔ Hexagon Socket Flat Countersunk Head Cap Screw - Inch 4-40 UNC x 0.25:14
- Insert:129: Deck_Bushing:10 ↔ Hexagon Socket Flat Countersunk Head Cap Screw - Inch 4-40 UNC x 0.25:13
- Insert:130: Deck_Bushing:1 ↔ Hexagon Socket Flat Countersunk Head Cap Screw - Inch 4-40 UNC x 0.25:16
- Insert:131: Deck_Bushing:10 ↔ Hexagon Socket Flat Countersunk Head Cap Screw - Inch 4-40 UNC x 0.25:15
- Insert:132: Deck_Bushing:3 ↔ Hexagon Socket Flat Countersunk Head Cap Screw - Inch 4-40 UNC x 0.25:18
- Insert:133: Deck_Bushing:9 ↔ Hexagon Socket Flat Countersunk Head Cap Screw - Inch 4-40 UNC x 0.25:17
- Insert:134: Deck_Bushing:3 ↔ Hexagon Socket Flat Countersunk Head Cap Screw - Inch 4-40 UNC x 0.25:20
- Insert:135: Deck_Bushing:9 ↔ Hexagon Socket Flat Countersunk Head Cap Screw - Inch 4-40 UNC x 0.25:19
- Mate:13: Deck_Bushing:9 ↔ Fender:1
- Insert:136: KWBH0001:1 ↔ Microswitch_Bracket:1
- Flush:2: KWBH0001:1 ↔ Microswitch_Bracket:1
- [Insert]: Internal Tooth Lock Washer - Type A (Inch) No. 4. Carbon Steel:1 ↔ Hexagon Socket Button Head Cap Screw - Inch 4 - 40 - 3/4:1
- Insert:138: Plain Washer (Inch) No. 4 - narrow - Type B:1 ↔ Internal Tooth Lock Washer - Type A (Inch) No. 4. Carbon Steel:1
- [Insert]: Internal Tooth Lock Washer - Type A (Inch) No. 4. Carbon Steel:2 ↔ Hexagon Socket Button Head Cap Screw - Inch 4 - 40 - 3/4:2
- [Insert]: Plain Washer (Inch) No. 4 - narrow - Type B:2 ↔ Internal Tooth Lock Washer - Type A (Inch) No. 4. Carbon Steel:2
- Insert:141: KWBH0001:1 ↔ Plain Washer (Inch) No. 4 - narrow - Type B:1
- Insert:142: KWBH0001:1 ↔ Plain Washer (Inch) No. 4 - narrow - Type B:2
- Mate:14: SCESCE-20N2010LP:1 ↔ Microswitch_Bracket:1
- Angle:1 (0 deg): SCESCE-20N2010LP:1 ↔ Microswitch_Bracket:1
- Mate:16 (127 mm): SCESCE-20N2010LP:1 ↔ Fender:1
- Mate:17: SCESCE-20N2010LP:1 ↔ Microswitch_Bracket:1
- [Insert]: Internal Tooth Lock Washer - Type A (Inch) No. 4. Carbon Steel:3 ↔ Hexagon Socket Button Head Cap Screw - Inch 4 - 40 - 3/4:3
- [Insert]: Plain Washer (Inch) No. 4 - narrow - Type B:3 ↔ Internal Tooth Lock Washer - Type A (Inch) No. 4. Carbon Steel:3
- [Insert]: Internal Tooth Lock Washer - Type A (Inch) No. 4. Carbon Steel:4 ↔ Hexagon Socket Button Head Cap Screw - Inch 4 - 40 - 3/4:4
- [Insert]: Plain Washer (Inch) No. 4 - narrow - Type B:4 ↔ Internal Tooth Lock Washer - Type A (Inch) No. 4. Carbon Steel:4
- Insert:147: SCESCE-20N2010LP:1 ↔ Plain Washer (Inch) No. 4 - narrow - Type B:3
- Insert:148: SCESCE-20N2010LP:1 ↔ Plain Washer (Inch) No. 4 - narrow - Type B:4
- [Insert]: KWBH0001:2 ↔ Microswitch_Bracket:2
- [Flush]: KWBH0001:2 ↔ Microswitch_Bracket:2
- [Insert]: Internal Tooth Lock Washer - Type A (Inch) No. 4. Carbon Steel:5 ↔ Hexagon Socket Button Head Cap Screw - Inch 4 - 40 - 3/4:5
- [Insert]: Plain Washer (Inch) No. 4 - narrow - Type B:5 ↔ Internal Tooth Lock Washer - Type A (Inch) No. 4. Carbon Steel:5
- [Insert]: Internal Tooth Lock Washer - Type A (Inch) No. 4. Carbon Steel:6 ↔ Hexagon Socket Button Head Cap Screw - Inch 4 - 40 - 3/4:6
- [Insert]: Plain Washer (Inch) No. 4 - narrow - Type B:6 ↔ Internal Tooth Lock Washer - Type A (Inch) No. 4. Carbon Steel:6
- [Insert]: KWBH0001:2 ↔ Plain Washer (Inch) No. 4 - narrow - Type B:5
- [Insert]: KWBH0001:2 ↔ Plain Washer (Inch) No. 4 - narrow - Type B:6
- [Insert]: Internal Tooth Lock Washer - Type A (Inch) No. 4. Carbon Steel:7 ↔ Hexagon Socket Button Head Cap Screw - Inch 4 - 40 - 3/4:7
- [Insert]: Plain Washer (Inch) No. 4 - narrow - Type B:7 ↔ Internal Tooth Lock Washer - Type A (Inch) No. 4. Carbon Steel:7
- [Insert]: Internal Tooth Lock Washer - Type A (Inch) No. 4. Carbon Steel:8 ↔ Hexagon Socket Button Head Cap Screw - Inch 4 - 40 - 3/4:8
- [Insert]: Plain Washer (Inch) No. 4 - narrow - Type B:8 ↔ Internal Tooth Lock Washer - Type A (Inch) No. 4. Carbon Steel:8
- [Insert]: KWBH0001:3 ↔ Microswitch_Bracket:3
- [Flush]: KWBH0001:3 ↔ Microswitch_Bracket:3
- [Insert]: Internal Tooth Lock Washer - Type A (Inch) No. 4. Carbon Steel:9 ↔ Hexagon Socket Button Head Cap Screw - Inch 4 - 40 - 3/4:9
- [Insert]: Plain Washer (Inch) No. 4 - narrow - Type B:9 ↔ Internal Tooth Lock Washer - Type A (Inch) No. 4. Carbon Steel:9
- [Insert]: Internal Tooth Lock Washer - Type A (Inch) No. 4. Carbon Steel:10 ↔ Hexagon Socket Button Head Cap Screw - Inch 4 - 40 - 3/4:10
- [Insert]: Plain Washer (Inch) No. 4 - narrow - Type B:10 ↔ Internal Tooth Lock Washer - Type A (Inch) No. 4. Carbon Steel:10
- [Insert]: KWBH0001:3 ↔ Plain Washer (Inch) No. 4 - narrow - Type B:9
- [Insert]: KWBH0001:3 ↔ Plain Washer (Inch) No. 4 - narrow - Type B:10
- [Insert]: Internal Tooth Lock Washer - Type A (Inch) No. 4. Carbon Steel:11 ↔ Hexagon Socket Button Head Cap Screw - Inch 4 - 40 - 3/4:11
- [Insert]: Plain Washer (Inch) No. 4 - narrow - Type B:11 ↔ Internal Tooth Lock Washer - Type A (Inch) No. 4. Carbon Steel:11
- [Insert]: Internal Tooth Lock Washer - Type A (Inch) No. 4. Carbon Steel:12 ↔ Hexagon Socket Button Head Cap Screw - Inch 4 - 40 - 3/4:12
- [Insert]: Plain Washer (Inch) No. 4 - narrow - Type B:12 ↔ Internal Tooth Lock Washer - Type A (Inch) No. 4. Carbon Steel:12
- [Insert]: KWBH0001:4 ↔ Microswitch_Bracket:4
- [Flush]: KWBH0001:4 ↔ Microswitch_Bracket:4
- [Insert]: Internal Tooth Lock Washer - Type A (Inch) No. 4. Carbon Steel:13 ↔ Hexagon Socket Button Head Cap Screw - Inch 4 - 40 - 3/4:13
- [Insert]: Plain Washer (Inch) No. 4 - narrow - Type B:13 ↔ Internal Tooth Lock Washer - Type A (Inch) No. 4. Carbon Steel:13
- [Insert]: Internal Tooth Lock Washer - Type A (Inch) No. 4. Carbon Steel:14 ↔ Hexagon Socket Button Head Cap Screw - Inch 4 - 40 - 3/4:14
- [Insert]: Plain Washer (Inch) No. 4 - narrow - Type B:14 ↔ Internal Tooth Lock Washer - Type A (Inch) No. 4. Carbon Steel:14
- [Insert]: KWBH0001:4 ↔ Plain Washer (Inch) No. 4 - narrow - Type B:13
- [Insert]: KWBH0001:4 ↔ Plain Washer (Inch) No. 4 - narrow - Type B:14
- [Insert]: Internal Tooth Lock Washer - Type A (Inch) No. 4. Carbon Steel:15 ↔ Hexagon Socket Button Head Cap Screw - Inch 4 - 40 - 3/4:15
- [Insert]: Plain Washer (Inch) No. 4 - narrow - Type B:15 ↔ Internal Tooth Lock Washer - Type A (Inch) No. 4. Carbon Steel:15
- [Insert]: Internal Tooth Lock Washer - Type A (Inch) No. 4. Carbon Steel:16 ↔ Hexagon Socket Button Head Cap Screw - Inch 4 - 40 - 3/4:16
- [Insert]: Plain Washer (Inch) No. 4 - narrow - Type B:16 ↔ Internal Tooth Lock Washer - Type A (Inch) No. 4. Carbon Steel:16
- [Insert]: KWBH0001:5 ↔ Microswitch_Bracket:5
- [Flush]: KWBH0001:5 ↔ Microswitch_Bracket:5
- [Insert]: Internal Tooth Lock Washer - Type A (Inch) No. 4. Carbon Steel:17 ↔ Hexagon Socket Button Head Cap Screw - Inch 4 - 40 - 3/4:17
- [Insert]: Plain Washer (Inch) No. 4 - narrow - Type B:17 ↔ Internal Tooth Lock Washer - Type A (Inch) No. 4. Carbon Steel:17
- [Insert]: Internal Tooth Lock Washer - Type A (Inch) No. 4. Carbon Steel:18 ↔ Hexagon Socket Button Head Cap Screw - Inch 4 - 40 - 3/4:18
- [Insert]: Plain Washer (Inch) No. 4 - narrow - Type B:18 ↔ Internal Tooth Lock Washer - Type A (Inch) No. 4. Carbon Steel:18
- [Insert]: KWBH0001:5 ↔ Plain Washer (Inch) No. 4 - narrow - Type B:17
- [Insert]: KWBH0001:5 ↔ Plain Washer (Inch) No. 4 - narrow - Type B:18
- [Insert]: Internal Tooth Lock Washer - Type A (Inch) No. 4. Carbon Steel:19 ↔ Hexagon Socket Button Head Cap Screw - Inch 4 - 40 - 3/4:19
- [Insert]: Plain Washer (Inch) No. 4 - narrow - Type B:19 ↔ Internal Tooth Lock Washer - Type A (Inch) No. 4. Carbon Steel:19
- [Insert]: Internal Tooth Lock Washer - Type A (Inch) No. 4. Carbon Steel:20 ↔ Hexagon Socket Button Head Cap Screw - Inch 4 - 40 - 3/4:20
- [Insert]: Plain Washer (Inch) No. 4 - narrow - Type B:20 ↔ Internal Tooth Lock Washer - Type A (Inch) No. 4. Carbon Steel:20
- [Insert]: KWBH0001:6 ↔ Microswitch_Bracket:6
- [Flush]: KWBH0001:6 ↔ Microswitch_Bracket:6
- [Insert]: Internal Tooth Lock Washer - Type A (Inch) No. 4. Carbon Steel:21 ↔ Hexagon Socket Button Head Cap Screw - Inch 4 - 40 - 3/4:21
- [Insert]: Plain Washer (Inch) No. 4 - narrow - Type B:21 ↔ Internal Tooth Lock Washer - Type A (Inch) No. 4. Carbon Steel:21
- [Insert]: Internal Tooth Lock Washer - Type A (Inch) No. 4. Carbon Steel:22 ↔ Hexagon Socket Button Head Cap Screw - Inch 4 - 40 - 3/4:22
- [Insert]: Plain Washer (Inch) No. 4 - narrow - Type B:22 ↔ Internal Tooth Lock Washer - Type A (Inch) No. 4. Carbon Steel:22
- [Insert]: KWBH0001:6 ↔ Plain Washer (Inch) No. 4 - narrow - Type B:21
- [Insert]: KWBH0001:6 ↔ Plain Washer (Inch) No. 4 - narrow - Type B:22
- [Insert]: Internal Tooth Lock Washer - Type A (Inch) No. 4. Carbon Steel:23 ↔ Hexagon Socket Button Head Cap Screw - Inch 4 - 40 - 3/4:23
- [Insert]: Plain Washer (Inch) No. 4 - narrow - Type B:23 ↔ Internal Tooth Lock Washer - Type A (Inch) No. 4. Carbon Steel:23
- [Insert]: Internal Tooth Lock Washer - Type A (Inch) No. 4. Carbon Steel:24 ↔ Hexagon Socket Button Head Cap Screw - Inch 4 - 40 - 3/4:24
- [Insert]: Plain Washer (Inch) No. 4 - narrow - Type B:24 ↔ Internal Tooth Lock Washer - Type A (Inch) No. 4. Carbon Steel:24
- [Insert]: KWBH0001:7 ↔ Microswitch_Bracket:7
- [Flush]: KWBH0001:7 ↔ Microswitch_Bracket:7